# Autodesk Inventor assembly: motor_set01
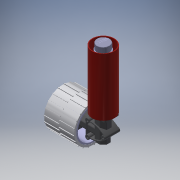
[picture p0: Inventor's stored thumbnail of the model, 180x180]
Saved by Autodesk Inventor 2018 (Build 220112000, 112)
## iProperties
Created: 2017-10-24
Part Number: motor_set01
Material: 一般
Document SubType Name: Assembly
Designer: 翔
Mass: 4283.24 g
Surface Area: 4489.39 cm^2
Volume: 2221.38 cm^3
Density: 1.92818 g/cm^3
Author: 翔
## Documents named in this file (6)
- E:\forest_robot_cad\Forest_v4\wheel\motor_set01.iam
- E:\forest_robot_cad\Forest_v4\wheel\DCmotor40W.iam
- E:\forest_robot_cad\Forest_v4\khk_KBX-151L\KBX-151L.ipt
- E:\forest_robot_cad\Forest_v4\wheel\tire_out.iam
- E:\forest_robot_cad\Forest_v4\wheel\Hub_v4.ipt
- E:\forest_robot_cad\Forest_v4\wheel\motor_cover_sample.ipt
## Components (5 placed, 5 different names)
1. DCmotor40W:1 [sub-assembly] — メイト:2, メイト:3, メイト:10
2. KBX-151L:1 — メイト:1, メイト:2, メイト:3, メイト:4, メイト:5, メイト:9, メイト:11
3. tire_out:1 [sub-assembly] — メイト:1, メイト:6, メイト:7, メイト:8
4. Hub_v4:1 — メイト:4, メイト:5, メイト:6, メイト:7, メイト:8, メイト:9
5. motor_cover_sample:1 — メイト:10, メイト:11
## Relationships (11: Mate 11)
- メイト:1 [Mate]: KBX-151L:1 ↔ tire_out:1
- メイト:2 [Mate]: DCmotor40W:1 ↔ KBX-151L:1
- メイト:3 [Mate]: DCmotor40W:1 ↔ KBX-151L:1
- メイト:4 [Mate]: KBX-151L:1 ↔ Hub_v4:1
- メイト:5 [Mate]: KBX-151L:1 ↔ Hub_v4:1
- メイト:6 [Mate]: tire_out:1 ↔ Hub_v4:1
- メイト:7 [Mate]: tire_out:1 ↔ Hub_v4:1
- メイト:8 [Mate]: tire_out:1 ↔ Hub_v4:1
- メイト:9 [Mate]: KBX-151L:1 ↔ Hub_v4:1
- メイト:10 [Mate]: DCmotor40W:1 ↔ motor_cover_sample:1
- メイト:11 [Mate]: KBX-151L:1 ↔ motor_cover_sample:1
